# Autodesk Inventor assembly: whole_assembly
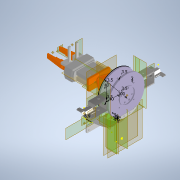
[picture p0: Inventor's stored thumbnail of the model, 180x180]
Saved by Autodesk Inventor 2021 (Build 250183000, 183)
## iProperties
Created: 2023-03-20
Part Number: whole_assembly
Document SubType Name: Assembly
Designer: mahmo
Author: mahmo
## Documents named in this file (9)
- D:\new_gripper\whole_assembly.iam
- D:\new_gripper\3dfindit-Festo-539636_HGP-16-A-B-SSK---_asm_0_-ZH_-0202303061711339323165410e898ce\AIS2021\539636 HGP-16-A-B-SSK---(asm_0_-ZH).iam
- D:\new_gripper\tool_holder.ipt
- D:\new_gripper\Part3.ipt
- D:\new_gripper\suction_cup_holder.ipt
- D:\new_gripper\manga.ipt
- D:\new_gripper\normal_finger.ipt
- D:\new_gripper\reverse_finger.ipt
- D:\new_gripper\d435 i\Intel Realsense D435.ipt
## Components (11 placed, 8 different names)
1. 539636 HGP-16-A-B-SSK---(asm_0_-ZH):1 [sub-assembly] — Mate:1, Mate:2, Mate:7, Flush:4, Mate:23, Mate:24, Mate:25, Mate:26, Flush:5, Flush:8, Flush:9, Mate:37, Mate:38, Mate:39, Mate:40, Mate:47, Mate:59, Mate:62
2. tool_holder:1 — Mate:1, Mate:2, Mate:3, Mate:6, Flush:1, Mate:18, Mate:20, Mate:21, Mate:22, Mate:35, Mate:36
3. Part3:1 — Mate:3, Mate:6, Flush:1, Mate:7, Mate:17, Mate:19, Mate:29, Mate:34, Flush:10, Mate:45
4. suction_cup_holder:1 — Mate:17, Mate:18, Mate:19, Mate:48, Mate:49
5. manga:1 — Mate:20, Mate:21, Mate:22, Mate:64, Angle:1, Mate:65
6. normal_finger:1 — Flush:4, Mate:23, Mate:24, Mate:41
7. normal_finger:2 — Mate:25, Mate:26, Flush:5, Mate:42, Flush:11, Flush:12
8. suction_cup_holder:2 — Mate:29, Mate:34, Mate:35, Mate:43, Mate:44
9. reverse_finger:1 — Mate:39, Mate:40, Mate:41
10. reverse_finger:2 — Mate:37, Mate:38, Mate:42
11. Intel Realsense D435:1 — Mate:64, Angle:1, Mate:65
## Relationships (49: Mate 40, Flush 8, Angle 1)
- Mate:1: 539636 HGP-16-A-B-SSK---(asm_0_-ZH):1 ↔ tool_holder:1
- Mate:2: 539636 HGP-16-A-B-SSK---(asm_0_-ZH):1 ↔ tool_holder:1
- Mate:3: tool_holder:1 ↔ Part3:1
- Mate:6: tool_holder:1 ↔ Part3:1
- Flush:1: tool_holder:1 ↔ Part3:1
- Mate:7: 539636 HGP-16-A-B-SSK---(asm_0_-ZH):1 ↔ Part3:1
- Mate:17: Part3:1 ↔ suction_cup_holder:1
- Mate:18: tool_holder:1 ↔ suction_cup_holder:1
- Mate:19: Part3:1 ↔ suction_cup_holder:1
- Mate:20: tool_holder:1 ↔ manga:1
- Mate:21: tool_holder:1 ↔ manga:1
- Mate:22: tool_holder:1 ↔ manga:1
- Flush:4: 539636 HGP-16-A-B-SSK---(asm_0_-ZH):1 ↔ normal_finger:1
- Mate:23: 539636 HGP-16-A-B-SSK---(asm_0_-ZH):1 ↔ normal_finger:1
- Mate:24: 539636 HGP-16-A-B-SSK---(asm_0_-ZH):1 ↔ normal_finger:1
- Mate:25: 539636 HGP-16-A-B-SSK---(asm_0_-ZH):1 ↔ normal_finger:2
- Mate:26: 539636 HGP-16-A-B-SSK---(asm_0_-ZH):1 ↔ normal_finger:2
- Flush:5: 539636 HGP-16-A-B-SSK---(asm_0_-ZH):1 ↔ normal_finger:2
- Mate:29: Part3:1 ↔ suction_cup_holder:2
- Mate:34: Part3:1 ↔ suction_cup_holder:2
- Mate:35: tool_holder:1 ↔ suction_cup_holder:2
- Mate:36: tool_holder:1
- Flush:8: 539636 HGP-16-A-B-SSK---(asm_0_-ZH):1
- Flush:9: 539636 HGP-16-A-B-SSK---(asm_0_-ZH):1
- Flush:10: Part3:1
- Mate:37: 539636 HGP-16-A-B-SSK---(asm_0_-ZH):1 ↔ reverse_finger:2
- Mate:38: 539636 HGP-16-A-B-SSK---(asm_0_-ZH):1 ↔ reverse_finger:2
- Mate:39: 539636 HGP-16-A-B-SSK---(asm_0_-ZH):1 ↔ reverse_finger:1
- Mate:40: 539636 HGP-16-A-B-SSK---(asm_0_-ZH):1 ↔ reverse_finger:1
- Mate:41: normal_finger:1 ↔ reverse_finger:1
- Mate:42: normal_finger:2 ↔ reverse_finger:2
- Mate:43: suction_cup_holder:2
- Mate:44: suction_cup_holder:2
- Mate:45: Part3:1
- Mate:46
- Mate:47: 539636 HGP-16-A-B-SSK---(asm_0_-ZH):1
- Mate:48: suction_cup_holder:1
- Mate:49: suction_cup_holder:1
- Mate:53
- Flush:11: normal_finger:2
- Flush:12: normal_finger:2
- Mate:57
- Mate:58
- Mate:59: 539636 HGP-16-A-B-SSK---(asm_0_-ZH):1
- Mate:60
- Mate:62: 539636 HGP-16-A-B-SSK---(asm_0_-ZH):1
- Mate:64: manga:1 ↔ Intel Realsense D435:1
- Angle:1 (0 deg): manga:1 ↔ Intel Realsense D435:1
- Mate:65: manga:1 ↔ Intel Realsense D435:1
